# Autodesk Inventor assembly: łaziik
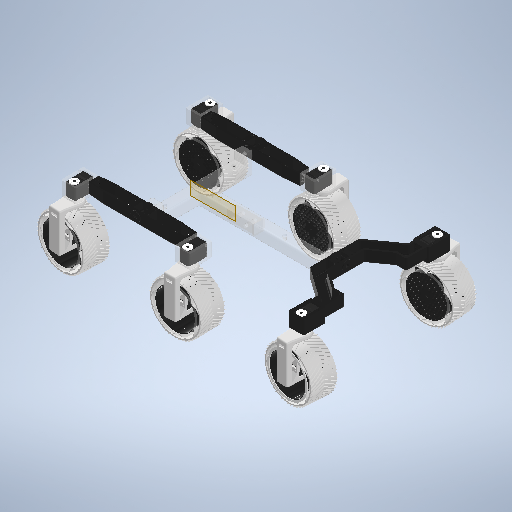
[picture p0: Inventor's stored thumbnail of the model, 512x512]
Saved by Autodesk Inventor 2025.3 (Build 293356000, 356)
## iProperties
Created: 2026-05-13
Part Number: łaziik
Document SubType Name: Assembly
Designer: ksawe
Author: ksawe
## Documents named in this file (5)
- C:\Users\ksawe\OneDrive\Pulpit\Exomy v1\wersja3\łaziik.iam
- C:\Users\ksawe\OneDrive\Pulpit\Exomy v1\wersja3\e.ipt
- C:\Users\ksawe\OneDrive\Pulpit\Exomy v1\wersja3\L.ipt
- C:\Users\ksawe\OneDrive\Pulpit\Exomy v1\wersja3\kinematicassembly.iam
- C:\Users\ksawe\OneDrive\Pulpit\Exomy v1\wersja3\kinematicpairback.iam
## Components (5 placed, 4 different names)
1. e:1 — Rigid:1, Rotational:2, Rotational:3
2. L:1 — Rigid:1, Rotational:1
3. kinematicassembly:1 [sub-assembly] — Rotational:2
4. kinematicassembly:2 [sub-assembly] — Rotational:3
5. kinematicpairback:1 [sub-assembly] — Rotational:1
## Relationships (4: RevoluteJoint 3, WeldJoint 1)
- Rigid:1 [WeldJoint]: e:1 ↔ L:1
- Rotational:1 [RevoluteJoint]: L:1 ↔ kinematicpairback:1
- Rotational:2 [RevoluteJoint]: e:1 ↔ kinematicassembly:1
- Rotational:3 [RevoluteJoint]: e:1 ↔ kinematicassembly:2
